# Autodesk Inventor assembly: toe_joint
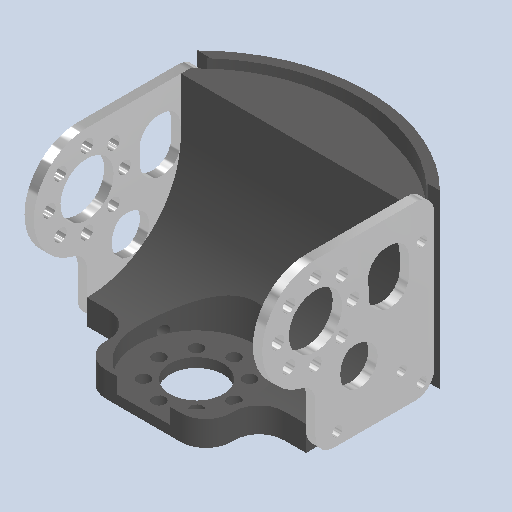
[picture p0: Inventor's stored thumbnail of the model, 512x512]
Saved by Autodesk Inventor 2026.1 (Build 301233020, 233B)
## iProperties
Created: 2024-02-11
Part Number: toe_joint
Document SubType Name: Assembly
Designer: hibik
Author: hibik
## Documents named in this file (3)
- C:\Users\hibik\Documents\Robomech\HR\Eglantyne_mark2\hard\leg\toe_joint.iam
- C:\Users\hibik\Documents\Robomech\HR\Eglantyne_mark2\hard\leg\toe_joint_middle.ipt
- C:\Users\hibik\Documents\Robomech\HR\Eglantyne_mark2\hard\leg\toe_joint.ipt
## Components (3 placed, 2 different names)
1. toe_joint_middle:1 — メイト:1, メイト:2, フラッシュ:1, フラッシュ:2, フラッシュ:3, フラッシュ:4
2. toe_joint:1 — メイト:2, フラッシュ:1, フラッシュ:4
3. toe_joint:2 — メイト:1, フラッシュ:2, フラッシュ:3
## Relationships (6: Flush 4, Mate 2)
- メイト:1 [Mate]: toe_joint_middle:1 ↔ toe_joint:2
- メイト:2 [Mate]: toe_joint_middle:1 ↔ toe_joint:1
- フラッシュ:1 [Flush]: toe_joint_middle:1 ↔ toe_joint:1
- フラッシュ:2 [Flush]: toe_joint_middle:1 ↔ toe_joint:2
- フラッシュ:3 [Flush]: toe_joint_middle:1 ↔ toe_joint:2
- フラッシュ:4 [Flush]: toe_joint_middle:1 ↔ toe_joint:1
